# Autodesk Inventor assembly: Leg Long
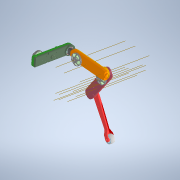
[picture p0: Inventor's stored thumbnail of the model, 180x180]
Saved by Autodesk Inventor 2022.2 (Build 262287000, 287)
## iProperties
Created: 2022-01-01
Part Number: Leg Long
Document SubType Name: Assembly
Designer: Jochen
Author: Jochen
## Documents named in this file (6)
- D:\Projects\Lisbeth\CAD\Leg Long.iam
- D:\Projects\Lisbeth\CAD\Thigh\Thigh.iam
- D:\Projects\Lisbeth\CAD\LowerLeg\LowerLeg.iam
- D:\Projects\Lisbeth\CAD\Hip\Hip.iam
- D:\Projects\Lisbeth\CAD\Lumbar\Lumbar.iam
- D:\Projects\Lisbeth\CAD\Hip\Hip Adapter.ipt
## Components (5 placed, 5 different names)
1. Thigh:1 [sub-assembly] — Mate:5, Mate:6, Mate:7, Mate:8
2. LowerLeg:1 [sub-assembly] — Mate:6, Mate:7
3. Hip:1 [sub-assembly] — Mate:3, Mate:4, Mate:5, Mate:8
4. Lumbar:1 [sub-assembly] — Mate:1, Mate:2
5. Hip Adapter:1 — Mate:1, Mate:2, Mate:3, Mate:4
## Relationships (8: Mate 8)
- Mate:1: Lumbar:1 ↔ Hip Adapter:1
- Mate:2: Lumbar:1 ↔ Hip Adapter:1
- Mate:3: Hip:1 ↔ Hip Adapter:1
- Mate:4: Hip:1 ↔ Hip Adapter:1
- Mate:5: Thigh:1 ↔ Hip:1
- Mate:6: Thigh:1 ↔ LowerLeg:1
- Mate:7: Thigh:1 ↔ LowerLeg:1
- Mate:8: Thigh:1 ↔ Hip:1
